# Autodesk Inventor assembly: Top Assembly
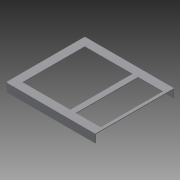
[picture p0: Inventor's stored thumbnail of the model, 180x180]
Saved by Autodesk Inventor 2015 (Build 190159000, 159)
## iProperties
Created: 2017-01-05
Part Number: Top Assembly
Document SubType Name: Weldment
Designer: ps2du
Weld Material: Welded Aluminum-6061
Author: ps2du
## Documents named in this file (5)
- E:\Robo Parts Inventor\Top Assembly.iam
- E:\Robo Parts Inventor\14in L Channel.ipt
- E:\Robo Parts Inventor\16in L Channel.ipt
- E:\Robo Parts Inventor\Top Front Steel Beam.ipt
- E:\Robo Parts Inventor\14in 1in flatstock.ipt
## Components (5 placed, 4 different names)
1. 14in L Channel:3 — Rigid:1, Rigid:4
2. 16in L Channel:1 — Rigid:1, Rigid:6
3. 16in L Channel:2 — Rigid:4, Rigid:5
4. Top Front Steel Beam:1 — Rigid:5
5. 14in 1in flatstock:1 — Rigid:6
## Relationships (4: WeldJoint 4)
- Rigid:1 [WeldJoint]: 14in L Channel:3 ↔ 16in L Channel:1
- Rigid:4 [WeldJoint]: 14in L Channel:3 ↔ 16in L Channel:2
- Rigid:5 [WeldJoint]: 16in L Channel:2 ↔ Top Front Steel Beam:1
- Rigid:6 [WeldJoint] (127 mm): 16in L Channel:1 ↔ 14in 1in flatstock:1
